# Autodesk Inventor assembly: Assembly1 Focusrite
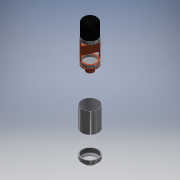
[picture p0: Inventor's stored thumbnail of the model, 180x180]
Saved by Autodesk Inventor 2018 (Build 220112000, 112)
## iProperties
Created: 2017-11-14
Part Number: Assembly1 Focusrite
Document SubType Name: Assembly
Designer: Justin
Author: Justin
## Documents named in this file (4)
- C:\Users\Justin\Documents\Assembly1 Focusrite.iam
- C:\Users\Justin\Documents\Part 1 of Focusrite Microphone.ipt
- C:\Users\Justin\Documents\Part 2 of Focusrite Microphone.ipt
- C:\Users\Justin\Documents\Part 3 of Focusrite Microphone.ipt
## Components (3 placed, 3 different names)
1. Part 1 of Focusrite Microphone:1 — Mate:1
2. Part 2 of Focusrite Microphone:1 — Mate:1, Mate:2
3. Part 3 of Focusrite Microphone:1 — Mate:2
## Relationships (2: Mate 2)
- Mate:1: Part 1 of Focusrite Microphone:1 ↔ Part 2 of Focusrite Microphone:1
- Mate:2: Part 2 of Focusrite Microphone:1 ↔ Part 3 of Focusrite Microphone:1
